# Autodesk Inventor assembly: Assembly_fuselage
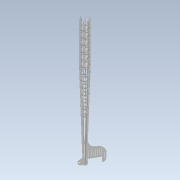
[picture p0: Inventor's stored thumbnail of the model, 180x180]
Saved by Autodesk Inventor 2020 (Build 240168000, 168)
## iProperties
Created: 2020-09-11
Part Number: Assembly_fuselage
Document SubType Name: Assembly
Designer: Admin
Author: Admin
## Documents named in this file (12)
- C:\PFE\Project_github\YFA-Project_python_interface\3D models\avion\Fuselage\Assembly_fuselage.iam
- C:\PFE\Project_github\YFA-Project_python_interface\3D models\avion\Fuselage\Rings\main_ring.ipt
- C:\PFE\Project_github\YFA-Project_python_interface\3D models\avion\Fuselage\Traverses fuselage\traverse_cote - top.ipt
- C:\PFE\Project_github\YFA-Project_python_interface\3D models\avion\Fuselage\Rings\Ring_n2.ipt
- C:\PFE\Project_github\YFA-Project_python_interface\3D models\avion\Fuselage\Rings\Ring_n3.ipt
- C:\PFE\Project_github\YFA-Project_python_interface\3D models\avion\Fuselage\Rings\Ring_n4.ipt
- C:\PFE\Project_github\YFA-Project_python_interface\3D models\avion\Fuselage\Rings\Ring_n5.ipt
- C:\PFE\Project_github\YFA-Project_python_interface\3D models\avion\Fuselage\Rings\Ring_n6.ipt
- C:\PFE\Project_github\YFA-Project_python_interface\3D models\avion\Fuselage\Rings\Ring_n7.ipt
- C:\PFE\Project_github\YFA-Project_python_interface\3D models\avion\Fuselage\Rings\Ring_n8.ipt
- C:\PFE\Project_github\YFA-Project_python_interface\3D models\avion\Fuselage\Traverses fuselage\traverse_cote - bottom.ipt
- C:\PFE\Project_github\YFA-Project_python_interface\3D models\avion\Fuselage\Traverses fuselage\traverse_cote.ipt
## Components (19 placed, 11 different names)
1. main_ring:1 — Mate:1, Mate:2, Mate:3, Mate:40, Mate:41, Mate:42, Mate:43, Mate:44, Mate:45, Mate:46, Mate:47, Mate:48, Mate:49, Mate:50, Mate:51, Mate:52, Mate:53, Mate:54
2. traverse_cote - top:1 — Mate:1, Mate:2, Mate:3, Mate:4, Mate:5, Mate:6, Mate:7, Mate:8, Mate:9, Mate:10, Mate:11, Mate:12, Mate:13, Mate:14, Mate:15, Mate:16, Mate:18, Mate:19, Mate:20, Mate:21, Mate:22, Mate:23, Mate:24, Mate:25, Mate:26, Mate:27, Mate:28, Mate:29, Mate:30, Mate:31, Mate:32, Mate:33, Mate:34, Mate:35, Mate:36, Mate:37, Mate:38, Mate:39
3. main_ring:2 — Mate:4, Mate:5, Mate:6
4. main_ring:4 — Mate:7, Mate:8, Mate:9
5. main_ring:5 — Mate:10, Mate:11, Mate:12
6. main_ring:6 — Mate:13, Mate:14, Mate:15, Mate:17
7. main_ring:7 — Mate:16, Mate:17, Mate:18
8. Ring_n2:1 — Mate:19, Mate:20, Mate:21
9. Ring_n3:1 — Mate:22, Mate:23, Mate:24
10. Ring_n4:1 — Mate:25, Mate:26, Mate:27
11. Ring_n5:1 — Mate:28, Mate:29, Mate:30
12. Ring_n6:1 — Mate:31, Mate:32, Mate:33
13. Ring_n7:1 — Mate:34, Mate:35, Mate:36
14. Ring_n8:1 — Mate:37, Mate:38, Mate:39
15. traverse_cote - bottom:1 — Mate:40, Mate:41, Mate:42
16. traverse_cote:1 — Mate:43, Mate:44, Mate:45
17. traverse_cote:2 — Mate:46, Mate:47, Mate:48
18. traverse_cote:3 — Mate:49, Mate:50, Mate:51
19. traverse_cote:4 — Mate:52, Mate:53, Mate:54
## Relationships (54: Mate 54)
- Mate:1: main_ring:1 ↔ traverse_cote - top:1
- Mate:2: main_ring:1 ↔ traverse_cote - top:1
- Mate:3: main_ring:1 ↔ traverse_cote - top:1
- Mate:4: traverse_cote - top:1 ↔ main_ring:2
- Mate:5: traverse_cote - top:1 ↔ main_ring:2
- Mate:6: traverse_cote - top:1 ↔ main_ring:2
- Mate:7: traverse_cote - top:1 ↔ main_ring:4
- Mate:8: traverse_cote - top:1 ↔ main_ring:4
- Mate:9: traverse_cote - top:1 ↔ main_ring:4
- Mate:10: traverse_cote - top:1 ↔ main_ring:5
- Mate:11: traverse_cote - top:1 ↔ main_ring:5
- Mate:12: traverse_cote - top:1 ↔ main_ring:5
- Mate:13: traverse_cote - top:1 ↔ main_ring:6
- Mate:14: traverse_cote - top:1 ↔ main_ring:6
- Mate:15: traverse_cote - top:1 ↔ main_ring:6
- Mate:16: traverse_cote - top:1 ↔ main_ring:7
- Mate:17: main_ring:6 ↔ main_ring:7
- Mate:18: traverse_cote - top:1 ↔ main_ring:7
- Mate:19: traverse_cote - top:1 ↔ Ring_n2:1
- Mate:20: traverse_cote - top:1 ↔ Ring_n2:1
- Mate:21: traverse_cote - top:1 ↔ Ring_n2:1
- Mate:22: traverse_cote - top:1 ↔ Ring_n3:1
- Mate:23: traverse_cote - top:1 ↔ Ring_n3:1
- Mate:24: traverse_cote - top:1 ↔ Ring_n3:1
- Mate:25: traverse_cote - top:1 ↔ Ring_n4:1
- Mate:26: traverse_cote - top:1 ↔ Ring_n4:1
- Mate:27: traverse_cote - top:1 ↔ Ring_n4:1
- Mate:28: traverse_cote - top:1 ↔ Ring_n5:1
- Mate:29: traverse_cote - top:1 ↔ Ring_n5:1
- Mate:30: traverse_cote - top:1 ↔ Ring_n5:1
- Mate:31: traverse_cote - top:1 ↔ Ring_n6:1
- Mate:32: traverse_cote - top:1 ↔ Ring_n6:1
- Mate:33: traverse_cote - top:1 ↔ Ring_n6:1
- Mate:34: traverse_cote - top:1 ↔ Ring_n7:1
- Mate:35: traverse_cote - top:1 ↔ Ring_n7:1
- Mate:36: traverse_cote - top:1 ↔ Ring_n7:1
- Mate:37: traverse_cote - top:1 ↔ Ring_n8:1
- Mate:38: traverse_cote - top:1 ↔ Ring_n8:1
- Mate:39: traverse_cote - top:1 ↔ Ring_n8:1
- Mate:40: main_ring:1 ↔ traverse_cote - bottom:1
- Mate:41: main_ring:1 ↔ traverse_cote - bottom:1
- Mate:42: main_ring:1 ↔ traverse_cote - bottom:1
- Mate:43: main_ring:1 ↔ traverse_cote:1
- Mate:44: main_ring:1 ↔ traverse_cote:1
- Mate:45: main_ring:1 ↔ traverse_cote:1
- Mate:46: main_ring:1 ↔ traverse_cote:2
- Mate:47: main_ring:1 ↔ traverse_cote:2
- Mate:48: main_ring:1 ↔ traverse_cote:2
- Mate:49: main_ring:1 ↔ traverse_cote:3
- Mate:50: main_ring:1 ↔ traverse_cote:3
- Mate:51: main_ring:1 ↔ traverse_cote:3
- Mate:52: main_ring:1 ↔ traverse_cote:4
- Mate:53: main_ring:1 ↔ traverse_cote:4
- Mate:54: main_ring:1 ↔ traverse_cote:4
